# Autodesk Inventor assembly: Magnet Frame Straight for 4040 - Assembly
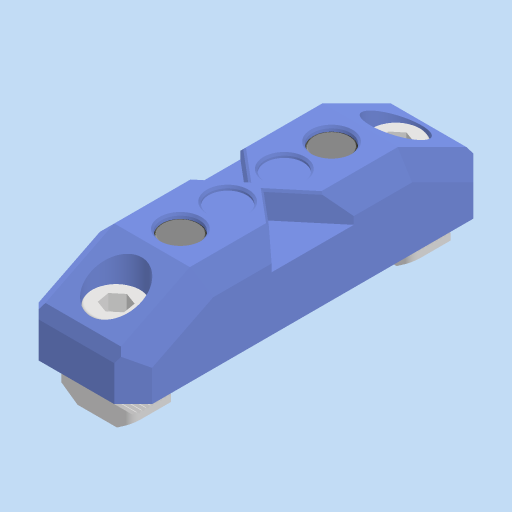
[picture p0: Inventor's stored thumbnail of the model, 512x512]
Saved by Autodesk Inventor 2023.2 (Build 272271000, 271)
## iProperties
Created: 2023-11-30
Part Number: Magnet Frame Straight for 4040 - Assembly
Document SubType Name: Assembly
Designer: Nils Bade
Author: Nils Bade
## Documents named in this file (5)
- C:\Users\nilsb\Documents\Inventor\Projektarbeit-Bade\Enclosure\Magnet Frame Straight for 4040 - Assembly.iam
- C:\Users\nilsb\Documents\Inventor\Projektarbeit-Bade\Enclosure\Magnet Frame straight for 4040.ipt
- C:\Users\nilsb\Documents\Inventor\Projektarbeit-Bade\Schrauben\Cap Head Screw M8x16 - DIN912.ipt
- C:\Users\nilsb\Documents\Inventor\Projektarbeit-Bade\Enclosure\Magnet-RatrigEnclosure.ipt
- C:\Users\nilsb\Documents\Inventor\Projektarbeit-Bade\RatRig_modified\T-NUT - DropIn 4040 SERIES - M8.ipt
## Components (7 placed, 4 different names)
1. Magnet Frame straight for 4040:1 — Passend:5, Passend:6, Passend:7, Passend:8, Passend:9, Passend:10, Passend:11, Passend:12, Winkel:1, Winkel:2, Passend:15, Passend:16
2. Cap Head Screw M8x16 - DIN912:1 — Passend:5, Passend:7, Passend:14
3. Cap Head Screw M8x16 - DIN912:2 — Passend:6, Passend:8, Passend:13
4. Magnet-RatrigEnclosure:1 — Passend:9, Passend:12
5. Magnet-RatrigEnclosure:2 — Passend:10, Passend:11
6. T-NUT - DROP IN TYPE FOR 40 SERIES - M8:1 — Passend:13, Winkel:2, Passend:16
7. T-NUT - DROP IN TYPE FOR 40 SERIES - M8:2 — Passend:14, Winkel:1, Passend:15
## Relationships (14: Mate 12, Angle 2)
- Passend:5 [Mate]: Magnet Frame straight for 4040:1 ↔ Cap Head Screw M8x16 - DIN912:1
- Passend:6 [Mate]: Magnet Frame straight for 4040:1 ↔ Cap Head Screw M8x16 - DIN912:2
- Passend:7 [Mate]: Magnet Frame straight for 4040:1 ↔ Cap Head Screw M8x16 - DIN912:1
- Passend:8 [Mate]: Magnet Frame straight for 4040:1 ↔ Cap Head Screw M8x16 - DIN912:2
- Passend:9 [Mate]: Magnet Frame straight for 4040:1 ↔ Magnet-RatrigEnclosure:1
- Passend:10 [Mate]: Magnet Frame straight for 4040:1 ↔ Magnet-RatrigEnclosure:2
- Passend:11 [Mate]: Magnet Frame straight for 4040:1 ↔ Magnet-RatrigEnclosure:2
- Passend:12 [Mate]: Magnet Frame straight for 4040:1 ↔ Magnet-RatrigEnclosure:1
- Passend:13 [Mate]: Cap Head Screw M8x16 - DIN912:2 ↔ T-NUT - DROP IN TYPE FOR 40 SERIES - M8:1
- Passend:14 [Mate]: Cap Head Screw M8x16 - DIN912:1 ↔ T-NUT - DROP IN TYPE FOR 40 SERIES - M8:2
- Winkel:1 [Angle] (0 deg): Magnet Frame straight for 4040:1 ↔ T-NUT - DROP IN TYPE FOR 40 SERIES - M8:2
- Winkel:2 [Angle] (0 deg): Magnet Frame straight for 4040:1 ↔ T-NUT - DROP IN TYPE FOR 40 SERIES - M8:1
- Passend:15 [Mate] (5.5 mm): Magnet Frame straight for 4040:1 ↔ T-NUT - DROP IN TYPE FOR 40 SERIES - M8:2
- Passend:16 [Mate] (5.5 mm): Magnet Frame straight for 4040:1 ↔ T-NUT - DROP IN TYPE FOR 40 SERIES - M8:1
